# Autodesk Inventor assembly: estufa morango 20
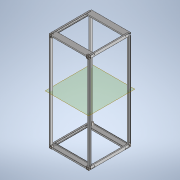
[picture p0: Inventor's stored thumbnail of the model, 180x180]
Saved by Autodesk Inventor 2020 (Build 240168000, 168)
## iProperties
Created: 2022-10-16
Part Number: estufa morango 20
Document SubType Name: Assembly
Designer: super
Author: super
## Documents named in this file (5)
- C:\desk\promissionsave\inventor\container\estufa morango 20.iam
- C:\desk\promissionsave\inventor\container\corners 20feet.iam
- C:\desk\promissionsave\inventor\container\c lateral struct.ipt
- C:\desk\promissionsave\inventor\container\pilar.ipt
- C:\desk\promissionsave\inventor\container\c trave.ipt
## Components (14 placed, 4 different names)
1. corners 20feet:1 [sub-assembly] — Mate:1, Mate:2, Flush:1, Mate:3, Flush:2, Flush:3, Mate:8, Flush:6, Flush:7, Flush:8, Flush:10
2. c lateral struct:1 — Mate:8, Flush:6, Flush:7
3. pilar:1 — Mate:3, Flush:2, Flush:5, Mate:7, Flush:8, Mate:10
4. c trave:1 — Flush:3, Flush:5, Mate:7, Flush:10
5. c lateral struct:2 — Mate:12
6. pilar:2
7. c trave:2
8. c lateral struct:3 — Mate:11
9. c lateral struct:4
10. c lateral struct:5 — Mate:13
11. pilar:3
12. c trave:3
13. pilar:4
14. c trave:4
## Relationships (19: Mate 9, Flush 9, Angle 1)
- Mate:1: corners 20feet:1
- Mate:2: corners 20feet:1
- Flush:1: corners 20feet:1
- Mate:3: corners 20feet:1 ↔ pilar:1
- Flush:2 (7 mm): corners 20feet:1 ↔ pilar:1
- Flush:3: corners 20feet:1 ↔ c trave:1
- Flush:5: pilar:1 ↔ c trave:1
- Mate:7: pilar:1 ↔ c trave:1
- Mate:8: corners 20feet:1 ↔ c lateral struct:1
- Flush:6 (7 mm): corners 20feet:1 ↔ c lateral struct:1
- Flush:7 (4 mm): corners 20feet:1 ↔ c lateral struct:1
- Flush:8: corners 20feet:1 ↔ pilar:1
- Mate:10: pilar:1
- Angle:1 (0 deg)
- Flush:9 (1219.2 mm)
- Flush:10 (4 mm): corners 20feet:1 ↔ c trave:1
- Mate:11: c lateral struct:3
- Mate:12: c lateral struct:2
- Mate:13: c lateral struct:5
